# Autodesk Inventor assembly: assem_linact_rod_v3
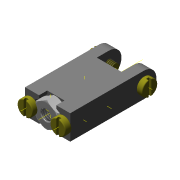
[picture p0: Inventor's stored thumbnail of the model, 180x180]
Saved by Autodesk Inventor 2014 (Build 180170000, 170)
## iProperties
Created: 2015-05-04
Part Number: assem_linact_rod_v3
Document SubType Name: Assembly
Designer: Martin
Author: Martin
## Documents named in this file (5)
- C:\Users\Martin\Dropbox\biohand-mec\biohand_v1\fingers\index\assem_linact_rod_v3.iam
- C:\Users\Martin\Dropbox\biohand-mec\biohand_v1\fingers\index\linact_rod_v3.ipt
- C:\Users\Martin\Dropbox\biohand-mec\biohand_v1\misc\m3_nut.ipt
- C:\Users\Martin\Dropbox\biohand-mec\biohand_v1\misc\m2_8_screw.ipt
- C:\Users\Martin\Dropbox\biohand-mec\biohand_v1\misc\m2_4_screw.ipt
## Components (6 placed, 4 different names)
1. linact_rod_v3:1 — Insert:1, Insert:2, Insert:3, Insert:4, Insert:5
2. m3_nut:1 — Insert:1, Angle:1
3. m2_8_screw:1 — Insert:2, Mate:1
4. m2_8_screw:2 — Insert:3, Mate:2
5. m2_4_screw:1 — Insert:4, Mate:3
6. m2_4_screw:2 — Insert:5, Mate:4
## Relationships (10: Insert 5, Mate 4, Angle 1)
- Insert:1: linact_rod_v3:1 ↔ m3_nut:1
- Angle:1 (90 deg): m3_nut:1
- Insert:2: linact_rod_v3:1 ↔ m2_8_screw:1
- Insert:3: linact_rod_v3:1 ↔ m2_8_screw:2
- Mate:1: m2_8_screw:1
- Mate:2: m2_8_screw:2
- Insert:4: linact_rod_v3:1 ↔ m2_4_screw:1
- Mate:3: m2_4_screw:1
- Insert:5: linact_rod_v3:1 ↔ m2_4_screw:2
- Mate:4: m2_4_screw:2
